# Autodesk Inventor assembly: A
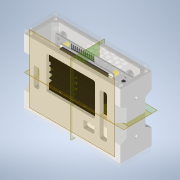
[picture p0: Inventor's stored thumbnail of the model, 180x180]
Saved by Autodesk Inventor 2022.2 (Build 262287000, 287)
## iProperties
Created: 2021-11-17
Part Number: A
Document SubType Name: Assembly
Designer: kfcs7
Author: kfcs7
## Documents named in this file (6)
- C:\Users\kfcs7\Desktop\Jetson-Nano-2GB-Case\A.iam
- C:\Users\kfcs7\Desktop\Jetson-Nano-2GB-Case\A-01.ipt
- C:\Users\kfcs7\Desktop\Jetson-Nano-2GB-Case\A-02.ipt
- C:\Users\kfcs7\Desktop\Jetson-Nano-2GB-Case\A-03.ipt
- C:\Users\kfcs7\3D Objects\Jetson Nano 2GB.iam
- C:\Users\kfcs7\Desktop\Jetson-Nano-2GB-Case\A-04.ipt
## Components (5 placed, 5 different names)
1. A-01:1 — Rigid:3, Rigid:1
2. A-02:1 — Rigid:3, Flush:1, Rigid:2
3. A-03:1 — Flush:1
4. Jetson Nano 2GB:1 [sub-assembly] — Rigid:1
5. A-04:1 — Rigid:2
## Relationships (4: WeldJoint 3, Flush 1)
- Rigid:3 [WeldJoint]: A-01:1 ↔ A-02:1
- Flush:1: A-02:1 ↔ A-03:1
- Rigid:1 [WeldJoint]: A-01:1 ↔ Jetson Nano 2GB:1
- Rigid:2 [WeldJoint]: A-02:1 ↔ A-04:1
